# Autodesk Inventor assembly: Wheel Orientation
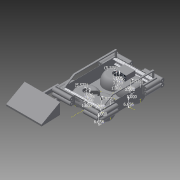
[picture p0: Inventor's stored thumbnail of the model, 180x180]
Saved by Autodesk Inventor 2015 (Build 190159000, 159)
## iProperties
Created: 2016-01-19
Part Number: Wheel Orientation
Document SubType Name: Assembly
Designer: sethbattis
Author: sethbattis
## Documents named in this file (11)
- \\area51\team3566\cad\FRC 2016\Space Claims.iam
- \\area51\team3566\cad\FRC 2016\Wheelbase.ipt
- \\area51\team3566\cad\FRC 2016\Snow Tire Wheel with Gearbox and CIM.ipt
- \\area51\team3566\cad\FRC 2016\Basic Frame.ipt
- \\area51\team3566\cad\FRC 2016\Corner Bumper.ipt
- \\area51\team3566\cad\FRC 2016\AM14U3 End Sheet 24.5in.ipt
- \\area51\team3566\cad\FRC 2016\Roll Bar.ipt
- \\area51\team3566\cad\FRC 2016\Floor.ipt
- \\area51\team3566\cad\FRC 2016\Imported Components\fc16-036_Battery.iam\fc16-036_Battery.iam.iam
- \\area51\team3566\cad\FRC 2016\Prow.ipt
- fc16-036_Battery.iam
## Components (17 placed, 9 different names)
1. Basic Frame:1 — Flush:1, Rigid:1, Mate:1, Mate:2, Flush:2, Flush:3, Flush:4, Flush:5, Mate:3, Mate:4, Flush:6, Flush:7, Flush:8, Flush:9, Mate:5, Flush:10, Mate:10, Mate:11, Mate:12, Flush:11, Flush:12, Flush:13, Flush:14, Flush:15, Rigid:2
2. Wheelbase:1 — Rotational:1, Rotational:2, Rotational:3, Rotational:4, Flush:1, Rigid:1
3. Snow Tire Wheel with Gearbox and CIM:1 — Rotational:2
4. Snow Tire Wheel with Gearbox and CIM:2 — Rotational:1
5. Snow Tire Wheel with Gearbox and CIM:3 — Rotational:4
6. Snow Tire Wheel with Gearbox and CIM:4 — Rotational:3
7. AM14U3 End Sheet 24.5in:1 — Flush:10, Mate:10
8. AM14U3 End Sheet 24.5in:2 — Mate:5, Mate:11
9. Roll Bar:1 — Flush:12, Flush:13, Flush:15
10. Roll Bar:2 — Mate:12, Flush:11, Flush:14
11. Floor:1 — Rigid:2, Mate:13
12. fc16-036_Battery.iam:1 [sub-assembly] — Mate:13
13. Prow:1
14. Corner Bumper:1 — Mate:1, Mate:3, Flush:6
15. Corner Bumper:2 — Mate:2, Flush:2, Flush:7
16. Corner Bumper:3 — Flush:4, Mate:4, Flush:9
17. Corner Bumper:4 — Flush:3, Flush:5, Flush:8
## Relationships (30: Flush 15, Mate 9, RevoluteJoint 4, WeldJoint 2)
- Rotational:1 [RevoluteJoint]: Wheelbase:1 ↔ Snow Tire Wheel with Gearbox and CIM:2
- Rotational:2 [RevoluteJoint]: Wheelbase:1 ↔ Snow Tire Wheel with Gearbox and CIM:1
- Rotational:3 [RevoluteJoint]: Wheelbase:1 ↔ Snow Tire Wheel with Gearbox and CIM:4
- Rotational:4 [RevoluteJoint]: Wheelbase:1 ↔ Snow Tire Wheel with Gearbox and CIM:3
- Flush:1: Basic Frame:1 ↔ Wheelbase:1
- Rigid:1 [WeldJoint]: Basic Frame:1 ↔ Wheelbase:1
- Mate:1: Basic Frame:1 ↔ Corner Bumper:1
- Mate:2: Basic Frame:1 ↔ Corner Bumper:2
- Flush:2: Basic Frame:1 ↔ Corner Bumper:2
- Flush:3: Basic Frame:1 ↔ Corner Bumper:4
- Flush:4: Basic Frame:1 ↔ Corner Bumper:3
- Flush:5: Basic Frame:1 ↔ Corner Bumper:4
- Mate:3: Basic Frame:1 ↔ Corner Bumper:1
- Mate:4: Basic Frame:1 ↔ Corner Bumper:3
- Flush:6: Basic Frame:1 ↔ Corner Bumper:1
- Flush:7: Basic Frame:1 ↔ Corner Bumper:2
- Flush:8: Basic Frame:1 ↔ Corner Bumper:4
- Flush:9: Basic Frame:1 ↔ Corner Bumper:3
- Mate:5: Basic Frame:1 ↔ AM14U3 End Sheet 24.5in:2
- Flush:10: Basic Frame:1 ↔ AM14U3 End Sheet 24.5in:1
- Mate:10: Basic Frame:1 ↔ AM14U3 End Sheet 24.5in:1
- Mate:11: Basic Frame:1 ↔ AM14U3 End Sheet 24.5in:2
- Mate:12: Basic Frame:1 ↔ Roll Bar:2
- Flush:11: Basic Frame:1 ↔ Roll Bar:2
- Flush:12: Basic Frame:1 ↔ Roll Bar:1
- Flush:13: Basic Frame:1 ↔ Roll Bar:1
- Flush:14: Basic Frame:1 ↔ Roll Bar:2
- Flush:15: Basic Frame:1 ↔ Roll Bar:1
- Rigid:2 [WeldJoint]: Basic Frame:1 ↔ Floor:1
- Mate:13: Floor:1 ↔ fc16-036_Battery.iam:1
